# Autodesk Inventor assembly: gun 2
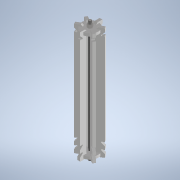
[picture p0: Inventor's stored thumbnail of the model, 180x180]
Saved by Autodesk Inventor 2020.1 (Build 241239000, 239)
## iProperties
Created: 2022-04-01
Part Number: gun 2
Document SubType Name: Assembly
Designer: User
Author: User
## Documents named in this file (4)
- D:\GitHub\TANK\3D-turret\gun 2.iam
- D:\GitHub\TANK\3D-turret\barrel_holder.ipt
- D:\GitHub\TANK\3D-turret\trunk 2.ipt
- D:\GitHub\TANK\3D-turret\ось пушки 2.ipt
## Components (9 placed, 3 different names)
1. barrel_holder:1 — Жесткий:1, С поворотом:1
2. barrel_holder:2 — Жесткий:2
3. ось пушки 2:1 — С поворотом:1
4. trunk 2:1 — Жесткий:1
5. trunk 2:7 — Жесткий:2
6. trunk 2:8
7. trunk 2:9
8. trunk 2:10
9. trunk 2:11
## Component patterns: (6 elements, first: trunk 2:1)
## Relationships (3: WeldJoint 2, RevoluteJoint 1)
- Жесткий:1 [WeldJoint]: barrel_holder:1 ↔ trunk 2:1
- Жесткий:2 [WeldJoint]: barrel_holder:2 ↔ trunk 2:7
- С поворотом:1 [RevoluteJoint]: barrel_holder:1 ↔ ось пушки 2:1
